# Autodesk Inventor assembly: MBRDAC45-2-10
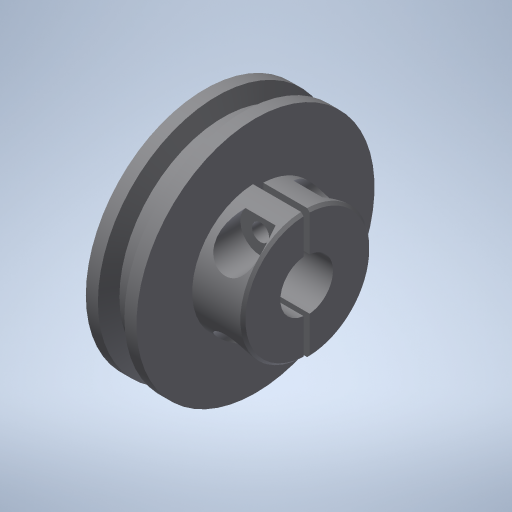
[picture p0: Inventor's stored thumbnail of the model, 512x512]
Saved by Autodesk Inventor 2024 (Build 280153000, 153)
## iProperties
Created: 2024-03-05
Part Number: MBRDAC45-2-10
Catalog Web Link: www.cadenas.de
Description: MBRDC, MBRDAC-Pulleys for Round Belts - Clamping Type - Trapezoid Groove
Vendor: MISUMI
Document SubType Name: Assembly
Designer: psAdmin
Manufacturer: MISUMI
Mass: 18.5371 g
Surface Area: 81.6751 cm^2
Volume: 18.5371 cm^3
Density: 1 g/cm^3
Category: PARTsolutions
Company: MISUMI
PSOL_IDENT_0: {$CADENAS_DATA/23d-libs/misumi/metric/52_belts_pulleys/mbrdc_asmtab.prj},203 {VTYP=3D},{STYP=ASSTAB}
PSOL_IDENT_1: ,{NB=MBRDAC45-2-10},{LINA=MBRDAC45-2-10},{NN=MBRDC, MBRDAC},{DATE=06.06.2021 23:11:25},{GEOMDATE=16.
PSOL_IDENT_2: 06.2016 00:32:00},{VERSION=},{LINEID=30},{WBVAR=MAT,PD,DDS},{WBNUMERIC=PD,DDS}  {NB=MBRDAC45-2-10},{
PSOL_IDENT_3: LINA=MBRDAC45-2-10},{KT=DUMMY},{PN=MBRDAC45-2-10},{TYPE=MBRDAC},{MAT=2},{ST=Clear Anodizing},{AC=Hex
PSOL_IDENT_4: agon Socket Head Cap Screw (x2) Stainless Steel},{PD=45},{PD0=23,28,30,40,45,48,60,80},{U=2.0},{DDS=
PSOL_IDENT_5: 10.00},{DS0=5,6,6.35,8,10,11,12},{D=25},{D1=47},{D2=41},{HH=2.0},{W=4.4},{L=20},{T=10},{LL=4.5},{X=9
PSOL_IDENT_6: .0},{Y=4.5},{M=M4},{CBD=4},{MM=4.000},{MMMIN=3.242},{DD1=8.0},{DD2=4.5},{PPATH=mbrdc/mbrdc_asmtpl.pr
PSOL_IDENT_7: j}
NB: MBRDAC45-2-10
NN: MBRDC, MBRDAC
NT: Pulleys for Round Belts - Clamping Type - Trapezoid Groove
NBSYN: $PN.
LINA: MBRDAC45-2-10
CATALOG: Misumi
PN: MBRDAC45-2-10
MAT: A5052
ST: Clear Anodizing
AC: Hexagon Socket Head Cap Screw (x2) Stainless Steel
PD: 45
U: 2
DDS: 10
D: 25
D1: 47
D2: 41
HH: 2
W: 4.4
L: 20
T: 10
LL: 4.5
X: 9
Y: 4.5
M: M4
CBD: 4
SUPPLIER: MISUMI
ARTICLENO: MBRDAC45-2-10
BOMINFO: MBRDAC45-2-10
CREATOR: CADENAS GmbH
Title: MBRDAC45-2-10
Author: Cadenas PARTsolutions
Comments: Pulleys for Round Belts - Clamping Type - Trapezoid Groove
## Documents named in this file (4)
- C:\Users\haruy\OneDrive - Kyushu University\KURT_工房共有\2023~2024\ハード\CAD\2024NHK\000_parts\タイミングベルト\AIS2024\MBRDAC45-2-10.iam
- C:\Users\haruy\OneDrive - Kyushu University\KURT_工房共有\2023~2024\ハード\CAD\2024NHK\000_parts\タイミングベルト\AIS2024\MBRDAC45-2-10_p1.ipt
- C:\Users\haruy\OneDrive - Kyushu University\KURT_工房共有\2023~2024\ハード\CAD\2024NHK\000_parts\タイミングベルト\AIS2024\MBRDAC45-2-10_p2.ipt
- C:\Users\haruy\OneDrive - Kyushu University\KURT_工房共有\2023~2024\ハード\CAD\2024NHK\000_parts\タイミングベルト\AIS2024\M4x10_p3.ipt
## Components (4 placed, 3 different names)
1. MBRDAC45-2-10_p1:1 — part1_to_part2_Z@1 <-> part2_to_part1_Z@2
2. MBRDAC45-2-10_p2:1 — part1_to_part2_Z@1 <-> part2_to_part1_Z@2, part2_to_screw1_Z@2 <-> IP1_Z@3, part2_to_screw2_Z@2 <-> IP1_Z@4
3. M4x10_p3:1 — part2_to_screw1_Z@2 <-> IP1_Z@3
4. M4x10_p3:2 — part2_to_screw2_Z@2 <-> IP1_Z@4
## Relationships (3: Mate 3)
- part1_to_part2_Z@1 <-> part2_to_part1_Z@2 [Mate]: MBRDAC45-2-10_p1:1 ↔ MBRDAC45-2-10_p2:1
- part2_to_screw1_Z@2 <-> IP1_Z@3 [Mate]: MBRDAC45-2-10_p2:1 ↔ M4x10_p3:1
- part2_to_screw2_Z@2 <-> IP1_Z@4 [Mate]: MBRDAC45-2-10_p2:1 ↔ M4x10_p3:2
